# Autodesk Inventor assembly: ASY PNS 1100 left module
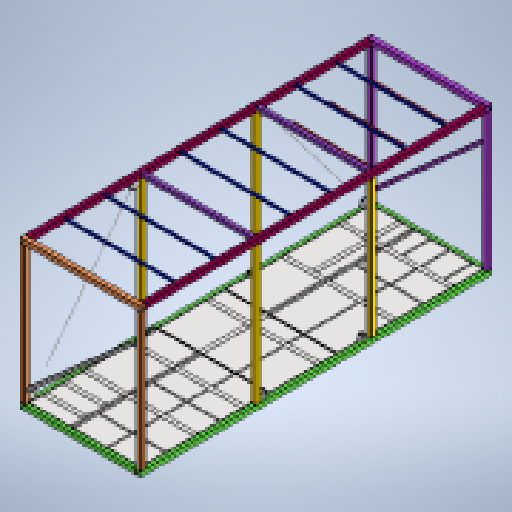
[picture p0: Inventor's stored thumbnail of the model, 512x512]
Saved by Autodesk Inventor 2025.3 (Build 293356030, 356C)
## iProperties
Created: 2025-03-25
Part Number: ASY PNS 1100 left module
Document SubType Name: Assembly
Designer: user
Mass: 1.00117e+06 g
Surface Area: 692723 cm^2
Volume: 127418 cm^3
Density: 7.85736 g/cm^3
Author: user
## Documents named in this file (11)
- C:\Users\admin\Yandex.Disk\home pc\Inventor\PNS2-Panaevsk\ASY PNS 1100 left module.iam
- C:\Users\admin\Yandex.Disk\home pc\Inventor\PNS2-Panaevsk\ASY PNS 1110 frame left floor.iam
- C:\Users\admin\Yandex.Disk\home pc\Inventor\PNS2-Panaevsk\ASY PNS 1120 frame featheredge.iam
- C:\Users\admin\Yandex.Disk\home pc\Inventor\PNS2-Panaevsk\ASY PNS 1130 frame featheredge.iam
- C:\Users\admin\Yandex.Disk\home pc\Inventor\PNS2-Panaevsk\PNS-0261 Upper beam.ipt
- C:\Users\admin\Yandex.Disk\home pc\Inventor\PNS2-Panaevsk\PNS-0262 middle pillar.ipt
- C:\Users\admin\Yandex.Disk\home pc\Inventor\PNS2-Panaevsk\PNS-071 stretch ring.ipt
- C:\Users\admin\Yandex.Disk\home pc\Inventor\PNS2-Panaevsk\PNS-0310 strench.ipt
- C:\Users\admin\Yandex.Disk\home pc\Inventor\PNS2-Panaevsk\PNS-0262 cross beam.ipt
- C:\Users\admin\Yandex.Disk\home pc\Inventor\PNS2-Panaevsk\PNS-0263 cross beam3.ipt
- C:\Users\admin\Yandex.Disk\home pc\Inventor\PNS2-Panaevsk\PNS-0264 cross channel.ipt
## Components (26 placed, 10 different names)
1. ASY PNS 1110 frame left floor:1 [sub-assembly]
2. ASY PNS 1120 frame featheredge:1 [sub-assembly] — Rigid:3, Rigid:4, Rigid:6, Rigid:7
3. ASY PNS 1130 frame featheredge:1 [sub-assembly] — Rigid:5, Rigid:8, Mate:12, Mate:13
4. PNS-0261 Upper beam:1 — Rigid:3, Mate:4, Flush:2, Mate:5, Flush:3, Mate:6, Flush:6, Mate:7, Mate:8, Mate:9, Mate:10, Mate:11, Flush:7, Flush:8, Flush:9, Flush:10, Flush:11
5. PNS-0261 Upper beam:2 — Rigid:4
6. PNS-0262 middle pillar:1 — Rigid:5, Flush:4
7. PNS-0262 middle pillar:2 — Rigid:8
8. PNS-0262 middle pillar:3 — Rigid:7
9. PNS-0262 middle pillar:4 — Rigid:6, Flush:5
10. PNS-071 stretch ring:1 — Mate:1, Flush:1
11. PNS-071 stretch ring:2
12. PNS-0310 strench:1 — Mate:1, Flush:1
13. PNS-071 stretch ring:3 — Mate:2, Mate:3
14. PNS-071 stretch ring:4
15. PNS-0310 strench:2 — Mate:2, Mate:3
16. PNS-0262 cross beam:1 — Mate:5, Flush:3, Flush:4, Mate:15, Mate:16, Mate:20, Flush:17
17. PNS-0262 cross beam:2 — Mate:4, Flush:2, Flush:5, Mate:17, Mate:18
18. PNS-0263 cross beam3:1 — Mate:6, Flush:6, Mate:18
19. PNS-0263 cross beam3:2 — Mate:7, Flush:11, Mate:17
20. PNS-0263 cross beam3:3 — Mate:8, Flush:10, Mate:16
21. PNS-0263 cross beam3:4 — Mate:9, Flush:9, Mate:15
22. PNS-0263 cross beam3:5 — Mate:10, Flush:8, Mate:13, Mate:19, Flush:18
23. PNS-0263 cross beam3:6 — Mate:11, Flush:7, Mate:12, Mate:14, Flush:16
24. PNS-0264 cross channel:1 — Mate:14, Flush:16
25. PNS-0264 cross channel:2 — Mate:20, Flush:17
26. PNS-0264 cross channel:3 — Mate:19, Flush:18
## Relationships (42: Mate 20, Flush 14, WeldJoint 8)
- [WeldJoint]: ASY PNS 1110 frame left floor:1 ↔ ASY PNS 1120 frame featheredge:1
- [WeldJoint]: ASY PNS 1110 frame left floor:1 ↔ ASY PNS 1130 frame featheredge:1
- Rigid:3 [WeldJoint] (-100 mm): ASY PNS 1120 frame featheredge:1 ↔ PNS-0261 Upper beam:1
- Rigid:4 [WeldJoint] (-100 mm): ASY PNS 1120 frame featheredge:1 ↔ PNS-0261 Upper beam:2
- Rigid:5 [WeldJoint] (2200 mm): ASY PNS 1130 frame featheredge:1 ↔ PNS-0262 middle pillar:1
- Rigid:6 [WeldJoint] (2200 mm): ASY PNS 1120 frame featheredge:1 ↔ PNS-0262 middle pillar:4
- Rigid:7 [WeldJoint] (2200 mm): ASY PNS 1120 frame featheredge:1 ↔ PNS-0262 middle pillar:3
- Rigid:8 [WeldJoint] (2200 mm): ASY PNS 1130 frame featheredge:1 ↔ PNS-0262 middle pillar:2
- Mate:1: PNS-071 stretch ring:1 ↔ PNS-0310 strench:1
- Flush:1: PNS-071 stretch ring:1 ↔ PNS-0310 strench:1
- Mate:2: PNS-071 stretch ring:3 ↔ PNS-0310 strench:2
- Mate:3: PNS-071 stretch ring:3 ↔ PNS-0310 strench:2
- Mate:4: PNS-0261 Upper beam:1 ↔ PNS-0262 cross beam:2
- Flush:2: PNS-0261 Upper beam:1 ↔ PNS-0262 cross beam:2
- Mate:5: PNS-0261 Upper beam:1 ↔ PNS-0262 cross beam:1
- Flush:3: PNS-0261 Upper beam:1 ↔ PNS-0262 cross beam:1
- Flush:4 (10 mm): PNS-0262 middle pillar:1 ↔ PNS-0262 cross beam:1
- Flush:5 (10 mm): PNS-0262 middle pillar:4 ↔ PNS-0262 cross beam:2
- Mate:6: PNS-0261 Upper beam:1 ↔ PNS-0263 cross beam3:1
- Flush:6: PNS-0261 Upper beam:1 ↔ PNS-0263 cross beam3:1
- Mate:7: PNS-0261 Upper beam:1 ↔ PNS-0263 cross beam3:2
- Mate:8: PNS-0261 Upper beam:1 ↔ PNS-0263 cross beam3:3
- Mate:9: PNS-0261 Upper beam:1 ↔ PNS-0263 cross beam3:4
- Mate:10: PNS-0261 Upper beam:1 ↔ PNS-0263 cross beam3:5
- Mate:11: PNS-0261 Upper beam:1 ↔ PNS-0263 cross beam3:6
- Flush:7: PNS-0261 Upper beam:1 ↔ PNS-0263 cross beam3:6
- Flush:8: PNS-0261 Upper beam:1 ↔ PNS-0263 cross beam3:5
- Flush:9: PNS-0261 Upper beam:1 ↔ PNS-0263 cross beam3:4
- Flush:10: PNS-0261 Upper beam:1 ↔ PNS-0263 cross beam3:3
- Flush:11: PNS-0261 Upper beam:1 ↔ PNS-0263 cross beam3:2
- Mate:12 (700 mm): ASY PNS 1130 frame featheredge:1 ↔ PNS-0263 cross beam3:6
- Mate:13 (1500 mm): ASY PNS 1130 frame featheredge:1 ↔ PNS-0263 cross beam3:5
- Mate:14: PNS-0263 cross beam3:6 ↔ PNS-0264 cross channel:1
- Flush:16: PNS-0263 cross beam3:6 ↔ PNS-0264 cross channel:1
- Mate:15 (700 mm): PNS-0262 cross beam:1 ↔ PNS-0263 cross beam3:4
- Mate:16 (1500 mm): PNS-0262 cross beam:1 ↔ PNS-0263 cross beam3:3
- Mate:17 (700 mm): PNS-0262 cross beam:2 ↔ PNS-0263 cross beam3:2
- Mate:18 (1500 mm): PNS-0262 cross beam:2 ↔ PNS-0263 cross beam3:1
- Mate:19: PNS-0263 cross beam3:5 ↔ PNS-0264 cross channel:3
- Mate:20: PNS-0262 cross beam:1 ↔ PNS-0264 cross channel:2
- Flush:17: PNS-0262 cross beam:1 ↔ PNS-0264 cross channel:2
- Flush:18: PNS-0263 cross beam3:5 ↔ PNS-0264 cross channel:3
